# Autodesk Inventor assembly: PowerDistroAssembly_RevC
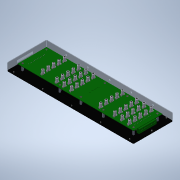
[picture p0: Inventor's stored thumbnail of the model, 180x180]
Saved by Autodesk Inventor 2020.2 (Build 242310000, 310)
## iProperties
Created: 2018-06-27
Part Number: PowerDistroAssembly_RevC
Document SubType Name: Assembly
Designer: Rich
Author: Rich
## Documents named in this file (6)
- C:\Users\Rich\development\UWaterloo\power-distro.git\SolidModels\PowerDistroAssembly_RevC.iam
- C:\Users\Rich\development\UWaterloo\power-distro.git\SolidModels\Enclosure2_RevB_Outer.ipt
- C:\Users\Rich\development\UWaterloo\power-distro.git\SolidModels\Enclosure2_RevB_Inner.ipt
- C:\Users\Rich\development\UWaterloo\power-distro.git\SolidModels\keystone-PN1608-2.ipt
- C:\Users\Rich\development\UWaterloo\power-distro.git\SolidModels\PowerDistroPCB_RevC.iam
- C:\Users\Rich\development\UWaterloo\power-distro.git\SolidModels\6-32x0.25 Slotted Flathead.ipt
## Components (35 placed, 5 different names)
1. Enclosure2_RevB_Outer:1 — Mate:30, Mate:34, Mate:35, Mate:36, Mate:37, Mate:38
2. Enclosure2_RevB_Inner:2 — Mate:30, Mate:37, Mate:38, Insert:1, Mate:39, Mate:40, Mate:41, Mate:42, Insert:7, Mate:46, Mate:47, Mate:48, Mate:49, Mate:50, Mate:51
3. PowerDistroPCB_RevC:1 [sub-assembly] — Mate:43, Mate:44, Mate:45, Insert:2, Insert:3, Insert:4, Insert:5, Insert:6
4. 6-32x0.25 Slotted Flathead:21 — Mate:50
5. 6-32x0.25 Slotted Flathead:22 — Mate:51
6. keystone-PN1608-2:1 — Insert:1, Mate:44
7. keystone-PN1608-2:2 — Mate:39
8. keystone-PN1608-2:3 — Mate:40
9. keystone-PN1608-2:4 — Mate:41
10. keystone-PN1608-2:5 — Mate:42
11. keystone-PN1608-2:6 — Mate:43, Mate:45
12. keystone-PN1608-2:7
13. keystone-PN1608-2:8
14. keystone-PN1608-2:9
15. keystone-PN1608-2:10
16. 6-32x0.25 Slotted Flathead:1 — Insert:2
17. 6-32x0.25 Slotted Flathead:2 — Insert:3
18. 6-32x0.25 Slotted Flathead:3 — Insert:4
19. 6-32x0.25 Slotted Flathead:4 — Insert:5
20. 6-32x0.25 Slotted Flathead:5 — Insert:6
21. 6-32x0.25 Slotted Flathead:6
22. 6-32x0.25 Slotted Flathead:7
23. 6-32x0.25 Slotted Flathead:8
24. 6-32x0.25 Slotted Flathead:9
25. 6-32x0.25 Slotted Flathead:10
26. 6-32x0.25 Slotted Flathead:11 — Insert:7
27. 6-32x0.25 Slotted Flathead:12 — Mate:49
28. 6-32x0.25 Slotted Flathead:13 — Mate:48
29. 6-32x0.25 Slotted Flathead:14 — Mate:47
30. 6-32x0.25 Slotted Flathead:15 — Mate:46
31. 6-32x0.25 Slotted Flathead:16
32. 6-32x0.25 Slotted Flathead:17
33. 6-32x0.25 Slotted Flathead:18
34. 6-32x0.25 Slotted Flathead:19
35. 6-32x0.25 Slotted Flathead:20
## Component patterns: (2 elements, first: keystone-PN1608-2:1 + keystone-PN1608-2:2 + keystone-PN1608-2:3 + keystone-PN1608-2:4 + keystone-PN1608-2:5), (2 elements, first: 6-32x0.25 Slotted Flathead:1 + 6-32x0.25 Slotted Flathead:2 + 6-32x0.25 Slotted Flathead:3 + 6-32x0.25 Slotted Flathead:4 + 6-32x0.25 Slotted Flathead:5), (2 elements, first: 6-32x0.25 Slotted Flathead:11 + 6-32x0.25 Slotted Flathead:12 + 6-32x0.25 Slotted Flathead:13 + 6-32x0.25 Slotted Flathead:14 + 6-32x0.25 Slotted Flathead:15)
## Relationships (26: Mate 19, Insert 7)
- Mate:30: Enclosure2_RevB_Outer:1 ↔ Enclosure2_RevB_Inner:2
- Mate:34: Enclosure2_RevB_Outer:1
- Mate:35: Enclosure2_RevB_Outer:1
- Mate:36: Enclosure2_RevB_Outer:1
- Mate:37: Enclosure2_RevB_Outer:1 ↔ Enclosure2_RevB_Inner:2
- Mate:38: Enclosure2_RevB_Outer:1 ↔ Enclosure2_RevB_Inner:2
- Insert:1: Enclosure2_RevB_Inner:2 ↔ keystone-PN1608-2:1
- Mate:39: Enclosure2_RevB_Inner:2 ↔ keystone-PN1608-2:2
- Mate:40: Enclosure2_RevB_Inner:2 ↔ keystone-PN1608-2:3
- Mate:41: Enclosure2_RevB_Inner:2 ↔ keystone-PN1608-2:4
- Mate:42: Enclosure2_RevB_Inner:2 ↔ keystone-PN1608-2:5
- Mate:43: PowerDistroPCB_RevC:1 ↔ keystone-PN1608-2:6
- Mate:44: PowerDistroPCB_RevC:1 ↔ keystone-PN1608-2:1
- Mate:45: PowerDistroPCB_RevC:1 ↔ keystone-PN1608-2:6
- Insert:2: PowerDistroPCB_RevC:1 ↔ 6-32x0.25 Slotted Flathead:1
- Insert:3: PowerDistroPCB_RevC:1 ↔ 6-32x0.25 Slotted Flathead:2
- Insert:4: PowerDistroPCB_RevC:1 ↔ 6-32x0.25 Slotted Flathead:3
- Insert:5: PowerDistroPCB_RevC:1 ↔ 6-32x0.25 Slotted Flathead:4
- Insert:6: PowerDistroPCB_RevC:1 ↔ 6-32x0.25 Slotted Flathead:5
- Insert:7: Enclosure2_RevB_Inner:2 ↔ 6-32x0.25 Slotted Flathead:11
- Mate:46: Enclosure2_RevB_Inner:2 ↔ 6-32x0.25 Slotted Flathead:15
- Mate:47: Enclosure2_RevB_Inner:2 ↔ 6-32x0.25 Slotted Flathead:14
- Mate:48: Enclosure2_RevB_Inner:2 ↔ 6-32x0.25 Slotted Flathead:13
- Mate:49: Enclosure2_RevB_Inner:2 ↔ 6-32x0.25 Slotted Flathead:12
- Mate:50: Enclosure2_RevB_Inner:2 ↔ 6-32x0.25 Slotted Flathead:21
- Mate:51: Enclosure2_RevB_Inner:2 ↔ 6-32x0.25 Slotted Flathead:22
